# Autodesk Inventor assembly: funnel_back_miirrored
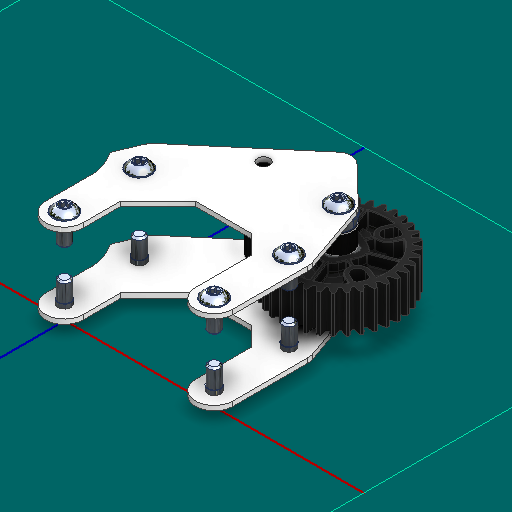
[picture p0: Inventor's stored thumbnail of the model, 512x512]
Saved by Autodesk Inventor 2025 (Build 290162000, 162)
## iProperties
Created: 2024-10-04
Part Number: funnel_back_miirrored
Document SubType Name: Assembly
Designer: Averey Ku
Author: Averey Ku
## Documents named in this file (16)
- C:\Users\avere\vex_robotics_high_stakes\hardware\cad\bots\high_stakes_v2\chassis\drivebay_mirrored\funnel_back_miirrored.iam
- C:\Users\avere\vex_robotics_high_stakes\hardware\cad\bots\high_stakes_v2\chassis\drivebay_mirrored\gusset_miirrored.ipt
- C:\Users\avere\vex_robotics_high_stakes\hardware\cad\robpros_cad_lib\Motion\Spacers\Washer Steel\SWasher .375 OD x .062500.ipt
- D:\vex_robotics_high_stakes\hardware\cad\robpros_cad_lib\Motion\Spacers\Washer Steel.ipt
- C:\Users\avere\vex_robotics_high_stakes\hardware\cad\bots\high_stakes_v2\chassis\drivebay_mirrored\Nut Keps_miirrored.ipt
- C:\Users\avere\vex_robotics_high_stakes\hardware\cad\robpros_cad_lib\Motion\Spacers\Spacer Nylon .375 OD\NSpacer .375 OD x .250.ipt
- D:\vex_robotics_high_stakes\hardware\cad\robpros_cad_lib\Motion\Spacers\Spacer Nylon .375 OD.ipt
- C:\Users\avere\vex_robotics_high_stakes\hardware\cad\robpros_cad_lib\Motion\Spacers\Washer Steel\SWasher .375 OD x .031250.ipt
- C:\Users\avere\vex_robotics_high_stakes\hardware\cad\VEX-CAD-Inventor\Structure\Hardware\Screw Steel - Star\SScrew Star Smooth .250.ipt
- D:\vex_robotics_high_stakes\hardware\cad\VEX-CAD-Inventor\Structure\Hardware\Screw Steel - Star.ipt
- C:\Users\avere\vex_robotics_high_stakes\hardware\cad\VEX-CAD-Inventor\Structure\Hardware\Screw Steel - Star\SScrew Star Smooth 1.250.ipt
- C:\Users\avere\vex_robotics_high_stakes\hardware\cad\bots\high_stakes_v2\chassis\drivebay_mirrored\Nut Hex_miirrored.ipt
- C:\Users\avere\vex_robotics_high_stakes\hardware\cad\VEX-CAD-Inventor\Structure\Hardware\Screw Shoulder Robosource\SScrew Shoulder Smooth .375 x .12.ipt
- D:\vex_robotics_high_stakes\hardware\cad\VEX-CAD-Inventor\Structure\Hardware\Screw Shoulder Robosource.ipt
- C:\Users\avere\vex_robotics_high_stakes\hardware\cad\bots\high_stakes_v2\chassis\drivebay_mirrored\HS 36T Gear, No Insert_miirrored.iam
- C:\Users\avere\vex_robotics_high_stakes\hardware\cad\robpros_cad_lib\Motion\Spacers\Spacer Nylon .375 OD\NSpacer .375 OD x .500.ipt
## Components (20 placed, 11 different names)
1. gusset_miirrored:1 — Mate:2, Insert:2, Insert:16, Insert:20, Insert:14, Insert:27
2. gusset_miirrored:2 — Angle:1, Mate:2, Insert:2, Mate:1, Insert:11, Insert:19, Insert:15
3. SWasher .375 OD x .062500:1 — Insert:9
4. Nut Keps_miirrored:1 — Insert:16, Insert:7
5. NSpacer .375 OD x .250:1 — Insert:7, Insert:25
6. SWasher .375 OD x .031250:2 — Insert:9
7. SScrew Star Smooth .250:1 — Insert:11
8. SScrew Star Smooth 1.250:2 — Insert:20
9. Nut Hex_miirrored:1 — Insert:19
10. HS 36T Gear, No Insert_miirrored:1 [sub-assembly] — Insert:25
11. NSpacer .375 OD x .500:2 — Insert:26
12. NSpacer .375 OD x .500:3 — Insert:27, Insert:26
13. SScrew Shoulder Smooth .375 x .12:1 — Insert:14
14. SScrew Shoulder Smooth .375 x .12:3
15. SScrew Shoulder Smooth .375 x .12:4
16. SScrew Shoulder Smooth .375 x .12:5
17. SScrew Shoulder Smooth .375 x .12:2 — Insert:15
18. SScrew Shoulder Smooth .375 x .12:6
19. SScrew Shoulder Smooth .375 x .12:7
20. SScrew Shoulder Smooth .375 x .12:8
## Component patterns: (4 elements, first: SScrew Shoulder Smooth .375 x .12:1), (4 elements, first: SScrew Shoulder Smooth .375 x .12:2)
## Relationships (15: Insert 12, Mate 2, Angle 1)
- Angle:1 (0 deg): gusset_miirrored:2
- Mate:2: gusset_miirrored:1 ↔ gusset_miirrored:2
- Insert:2 (25.4 mm): gusset_miirrored:1 ↔ gusset_miirrored:2
- Mate:1: gusset_miirrored:2
- Insert:16: gusset_miirrored:1 ↔ Nut Keps_miirrored:1
- Insert:7: Nut Keps_miirrored:1 ↔ NSpacer .375 OD x .250:1
- Insert:9: SWasher .375 OD x .062500:1 ↔ SWasher .375 OD x .031250:2
- Insert:11: gusset_miirrored:2 ↔ SScrew Star Smooth .250:1
- Insert:20: gusset_miirrored:1 ↔ SScrew Star Smooth 1.250:2
- Insert:19: gusset_miirrored:2 ↔ Nut Hex_miirrored:1
- Insert:14: gusset_miirrored:1 ↔ SScrew Shoulder Smooth .375 x .12:1
- Insert:15: gusset_miirrored:2 ↔ SScrew Shoulder Smooth .375 x .12:2
- Insert:25: NSpacer .375 OD x .250:1 ↔ HS 36T Gear, No Insert_miirrored:1
- Insert:27: gusset_miirrored:1 ↔ NSpacer .375 OD x .500:3
- Insert:26: NSpacer .375 OD x .500:2 ↔ NSpacer .375 OD x .500:3
